# Autodesk Inventor assembly: Krabicka
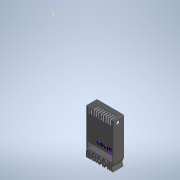
[picture p0: Inventor's stored thumbnail of the model, 180x180]
Saved by Autodesk Inventor 2021.2 (Build 252289000, 289)
## iProperties
Part Number: Krabicka
Document SubType Name: Sestava
Designer: herman
Author: herman
## Documents named in this file (5)
- C:\Users\Herman\ownCloud\Prace\Kicad\OndraMelodik\OndraMelodik\Krabicka.iam
- C:\Users\Herman\ownCloud\Prace\Kicad\OndraMelodik\OndraMelodik\Krabicka.ipt
- C:\Users\Herman\ownCloud\Prace\Kicad\OndraMelodik\OndraMelodik\Vicko.ipt
- C:\Users\Herman\ownCloud\Prace\Kicad\OndraMelodik\OndraMelodik\Deska.ipt
- C:\Users\Herman\ownCloud\Prace\Inventor\Projekty\Domek\Normalizovane soucasti\cs-CZ\ANSI B18.6.5M(22)\ANSI B18.6.5M - M2x0,4 x 6(38).ipt
## Components (5 placed, 4 different names)
1. Krabicka:1 — Stejný směr:1, Proti sobě:2
2. Vicko:1 — Stejný směr:1, Vložit:1, Vložit:2
3. Deska:1 — Proti sobě:2
4. Šroub samořezný s kónickou hlavou s křížovou drážkou - Typ D - Typ I - Metrický M2x0,4 x 6:1 — Vložit:1
5. Šroub samořezný s kónickou hlavou s křížovou drážkou - Typ D - Typ I - Metrický M2x0,4 x 6:2 — Vložit:2
## Relationships (4: Insert 2, Flush 1, Mate 1)
- Stejný směr:1 [Flush]: Krabicka:1 ↔ Vicko:1
- Proti sobě:2 [Mate]: Krabicka:1 ↔ Deska:1
- Vložit:1 [Insert]: Vicko:1 ↔ Šroub samořezný s kónickou hlavou s křížovou drážkou - Typ D - Typ I - Metrický M2x0,4 x 6:1
- Vložit:2 [Insert]: Vicko:1 ↔ Šroub samořezný s kónickou hlavou s křížovou drážkou - Typ D - Typ I - Metrický M2x0,4 x 6:2
